# Autodesk Inventor assembly: Organ Bank Pretty-Convex Assembly
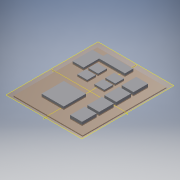
[picture p0: Inventor's stored thumbnail of the model, 180x180]
Saved by Autodesk Inventor 2019 (Build 230136000, 136)
## iProperties
Created: 2021-02-18
Part Number: Organ Bank Pretty-Convex Assembly
Document SubType Name: Assembly
Designer: Eric
Author: Eric
## Documents named in this file (7)
- C:\Users\Eric\Documents\! - Uni\Year 4\MENG-Robot-Fab-Project\Models\For_Optimiser\Organ Bank Assembly\Organ Bank Pretty-Convex Assembly.iam
- C:\Users\Eric\Documents\! - Uni\Year 4\MENG-Robot-Fab-Project\Models\For_Optimiser\Organ Bank Assembly\Convex Organ Bank Plate.ipt
- C:\Users\Eric\Documents\! - Uni\Year 4\MENG-Robot-Fab-Project\Models\For_Optimiser\Organ Bank Assembly\Convex Organ Bank Brain Slot.ipt
- C:\Users\Eric\Documents\! - Uni\Year 4\MENG-Robot-Fab-Project\Models\For_Optimiser\Organ Bank Assembly\Convex Organ Bank Castor Slots.ipt
- C:\Users\Eric\Documents\! - Uni\Year 4\MENG-Robot-Fab-Project\Models\For_Optimiser\Organ Bank Assembly\Convex Organ Bank Joint Slot.ipt
- C:\Users\Eric\Documents\! - Uni\Year 4\MENG-Robot-Fab-Project\Models\For_Optimiser\Organ Bank Assembly\Convex Organ Bank Motor Slot.ipt
- C:\Users\Eric\Documents\! - Uni\Year 4\MENG-Robot-Fab-Project\Models\For_Optimiser\Organ Bank Assembly\Convex Organ Bank Sensor Slot.ipt
## Components (12 placed, 6 different names)
1. Convex Organ Bank Plate:1 — Mate:2, Mate:3, Flush:8, Flush:9, Mate:6, Mate:10, Mate:11, Mate:12, Symmetry:1
2. Convex Organ Bank Brain Slot:1 — Symmetry:1
3. Convex Organ Bank Castor Slots:1 — Mate:2
4. Convex Organ Bank Joint Slot:1 — Mate:3
5. Convex Organ Bank Motor Slot:1
6. Convex Organ Bank Sensor Slot:1 — Mate:10
7. Convex Organ Bank Motor Slot:2
8. Convex Organ Bank Motor Slot:3 — Mate:6
9. Convex Organ Bank Motor Slot:4
10. Convex Organ Bank Sensor Slot:2 — Mate:11
11. Convex Organ Bank Sensor Slot:3
12. Convex Organ Bank Sensor Slot:4 — Mate:12
## Relationships (9: Mate 6, Flush 2, Symmetry 1)
- Mate:2: Convex Organ Bank Plate:1 ↔ Convex Organ Bank Castor Slots:1
- Mate:3: Convex Organ Bank Plate:1 ↔ Convex Organ Bank Joint Slot:1
- Flush:8: Convex Organ Bank Plate:1
- Flush:9: Convex Organ Bank Plate:1
- Mate:6: Convex Organ Bank Plate:1 ↔ Convex Organ Bank Motor Slot:3
- Mate:10: Convex Organ Bank Plate:1 ↔ Convex Organ Bank Sensor Slot:1
- Mate:11: Convex Organ Bank Plate:1 ↔ Convex Organ Bank Sensor Slot:2
- Mate:12: Convex Organ Bank Plate:1 ↔ Convex Organ Bank Sensor Slot:4
- Symmetry:1: Convex Organ Bank Plate:1 ↔ Convex Organ Bank Brain Slot:1
